# Autodesk Inventor assembly: Main Assembly
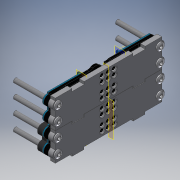
[picture p0: Inventor's stored thumbnail of the model, 180x180]
Saved by Autodesk Inventor 2016 (Build 200138000, 138)
## iProperties
Created: 2016-06-10
Part Number: Main Assembly
Document SubType Name: Assembly
Designer: Vijay
Author: Vijay
## Documents named in this file (6)
- C:\Users\Vijay\Dropbox\Personal\Refreshable Braille Display\Main Assembly.iam
- C:\Users\Vijay\Dropbox\Personal\Refreshable Braille Display\top.ipt
- C:\Users\Vijay\Dropbox\Personal\Refreshable Braille Display\Braille dots.ipt
- C:\Users\Vijay\Dropbox\Personal\Refreshable Braille Display\Cam pins.ipt
- C:\Users\Vijay\Dropbox\Personal\Refreshable Braille Display\Motor Holder combined.ipt
- C:\Users\Vijay\Documents\Inventor\Content Center Files\R2016\en-US\NF E 25-108 - A\NF E 25-108 - M2 x 20.ipt
## Components (19 placed, 5 different names)
1. top:1 — Angle:1, Flush:1, Mate:1, Mate:2, Mate:5, Mate:6, Mate:7, Mate:11, Mate:12, Mate:14, Rotational:5, Rotational:6, Rotational:7, Rotational:8, Mate:30, Angle:2
2. Braille dots:1 — Mate:3, Mate:4, Mate:8, Mate:21, Mate:22
3. top:2 — Angle:1, Flush:1, Mate:1, Mate:2, Mate:3, Mate:4, Mate:8, Mate:9, Mate:10, Mate:13, Rotational:1, Rotational:2, Rotational:3, Rotational:4
4. Braille dots:2 — Mate:9, Mate:10, Mate:13, Mate:15, Mate:16
5. Braille dots:3 — Mate:5, Mate:6, Mate:7, Mate:19, Mate:20, Mate:23
6. Braille dots:4 — Mate:11, Mate:12, Mate:14, Mate:17, Mate:18
7. Cam pins:1 — Mate:15, Mate:16, Flush:3
8. Cam pins:2 — Mate:21, Mate:22, Flush:2, Flush:4
9. Cam pins:3 — Mate:19, Mate:20, Flush:4, Mate:23
10. Cam pins:4 — Mate:17, Mate:18, Flush:2, Flush:3
11. NF E 25-108 - A M2 x 20:1 — Rotational:1, Mate:32
12. NF E 25-108 - A M2 x 20:2 — Rotational:3, Mate:31
13. NF E 25-108 - A M2 x 20:3 — Rotational:4
14. NF E 25-108 - A M2 x 20:4 — Rotational:2
15. NF E 25-108 - A M2 x 20:5 — Rotational:5
16. NF E 25-108 - A M2 x 20:6 — Rotational:6
17. NF E 25-108 - A M2 x 20:7 — Rotational:7
18. NF E 25-108 - A M2 x 20:8 — Rotational:8
19. Motor Holder combined:1 — Mate:31, Mate:32
## Relationships (40: Mate 26, RevoluteJoint 8, Flush 4, Angle 2)
- Angle:1 (180 deg): top:1 ↔ top:2
- Flush:1: top:1 ↔ top:2
- Mate:1 (0.11 mm): top:1 ↔ top:2
- Mate:2 (0.11 mm): top:1 ↔ top:2
- Mate:3: Braille dots:1 ↔ top:2
- Mate:4: Braille dots:1 ↔ top:2
- Mate:5: top:1 ↔ Braille dots:3
- Mate:6: top:1 ↔ Braille dots:3
- Mate:7: top:1 ↔ Braille dots:3
- Mate:8: Braille dots:1 ↔ top:2
- Mate:9: top:2 ↔ Braille dots:2
- Mate:10: top:2 ↔ Braille dots:2
- Mate:11: top:1 ↔ Braille dots:4
- Mate:12: top:1 ↔ Braille dots:4
- Mate:13: top:2 ↔ Braille dots:2
- Mate:14: top:1 ↔ Braille dots:4
- Mate:15: Braille dots:2 ↔ Cam pins:1
- Mate:16: Braille dots:2 ↔ Cam pins:1
- Mate:17: Braille dots:4 ↔ Cam pins:4
- Mate:18: Braille dots:4 ↔ Cam pins:4
- Mate:19: Braille dots:3 ↔ Cam pins:3
- Mate:20: Braille dots:3 ↔ Cam pins:3
- Mate:21: Braille dots:1 ↔ Cam pins:2
- Mate:22: Braille dots:1 ↔ Cam pins:2
- Flush:2: Cam pins:2 ↔ Cam pins:4
- Flush:3: Cam pins:1 ↔ Cam pins:4
- Flush:4: Cam pins:2 ↔ Cam pins:3
- Mate:23: Braille dots:3 ↔ Cam pins:3
- Rotational:1 [RevoluteJoint]: top:2 ↔ NF E 25-108 - A M2 x 20:1
- Rotational:2 [RevoluteJoint]: top:2 ↔ NF E 25-108 - A M2 x 20:4
- Rotational:3 [RevoluteJoint]: top:2 ↔ NF E 25-108 - A M2 x 20:2
- Rotational:4 [RevoluteJoint]: top:2 ↔ NF E 25-108 - A M2 x 20:3
- Rotational:5 [RevoluteJoint]: top:1 ↔ NF E 25-108 - A M2 x 20:5
- Rotational:6 [RevoluteJoint]: top:1 ↔ NF E 25-108 - A M2 x 20:6
- Rotational:7 [RevoluteJoint]: top:1 ↔ NF E 25-108 - A M2 x 20:7
- Rotational:8 [RevoluteJoint]: top:1 ↔ NF E 25-108 - A M2 x 20:8
- Mate:30: top:1
- Angle:2 (0 deg): top:1
- Mate:31: NF E 25-108 - A M2 x 20:2 ↔ Motor Holder combined:1
- Mate:32: NF E 25-108 - A M2 x 20:1 ↔ Motor Holder combined:1
